# Autodesk Inventor assembly: Shear 1 Assembly
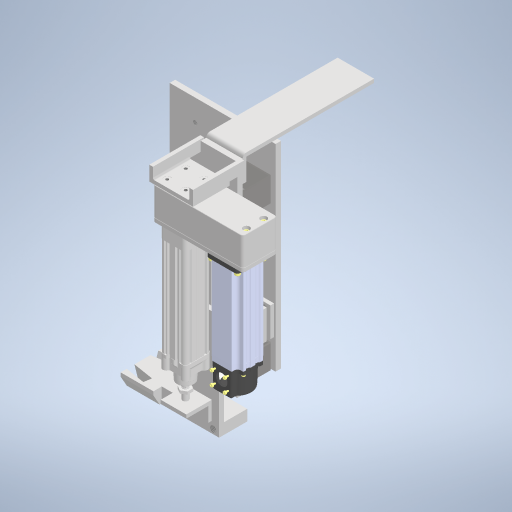
[picture p0: Inventor's stored thumbnail of the model, 512x512]
Saved by Autodesk Inventor 2024.2 (Build 282272000, 272)
## iProperties
Created: 2024-06-10
Part Number: Shear 1 Assembly
Document SubType Name: Assembly
Designer: AC91384
Author: AC91384
## Documents named in this file (12)
- K:\cadlib\1410\43A41410-2557\43A41410-2557.iam
- K:\cadlib\1410\43A41410-2557\Parts\Parts and Drawings\43A41410-2557a.ipt
- K:\cadlib\1410\43A41410-2557\Parts\Parts and Drawings\43A41410-2557B.ipt
- K:\cadlib\1410\43A41410-2557\Parts\Parts and Drawings\43A41410-2557D.ipt
- K:\cadlib\1410\43A41410-2557\Parts\Parts and Drawings\43A41410-2557C.ipt
- K:\cadlib\1410\43A41410-2557\Parts\Parts and Drawings\43A41410-2557Z.iam
- K:\cadlib\1410\43A41410-2557\Parts\Parts and Drawings\43A41410-2557I.ipt
- K:\cadlib\1410\43A41410-2557\Parts\Parts and Drawings\43A41410-2557H.ipt
- K:\cadlib\1410\43A41410-2557\Parts\Parts and Drawings\43A41410-2557F.ipt
- K:\cadlib\1410\43A41410-2557\Parts\Parts and Drawings\43A41410-2557E.ipt
- K:\cadlib\1410\43A41410-2557\Parts\Parts and Drawings\43A41410-2557G.ipt
- K:\cadlib\1410\43A41410-2557\Parts\Parts and Drawings\43A41410-2557J.ipt
## Components (12 placed, 11 different names)
1. 43A41410-2557a:1 — Mate:5, Flush:9, Flush:10, Flush:11, Mate:8, Mate:9, Flush:15, Mate:12, Flush:16, Mate:16, Flush:19, Mate:17, Flush:20
2. 43A41410-2557B:1 — Flush:3, Flush:4, Flush:5, Flush:6, Flush:7, Mate:2, Flush:8, Mate:4, Mate:15
3. 43A41410-2557D:1 — Flush:6, Flush:7, Mate:15
4. 43A41410-2557C:1 — Flush:3, Flush:4, Flush:5
5. 43A41410-2557Z:1 [sub-assembly] — Mate:2, Rotational:1
6. 43A41410-2557I:1 — Flush:8, Mate:4, Mate:5, Flush:9, Flush:10, Mate:11, Mate:14, Flush:18, Flush:21, Flush:22, Flush:23
7. 43A41410-2557H:1 — Flush:14, Mate:9, Flush:15
8. 43A41410-2557H:4 — Flush:11, Mate:8, Flush:14, Flush:23
9. 43A41410-2557F:1 — Mate:11, Rotational:1, Flush:21
10. 43A41410-2557E:1 — Mate:12, Flush:16, Flush:20
11. 43A41410-2557G:1 — Mate:14, Flush:18, Flush:22
12. 43A41410-2557J:1 — Mate:16, Flush:19, Mate:17
## Relationships (30: Flush 18, Mate 11, RevoluteJoint 1)
- Flush:3: 43A41410-2557B:1 ↔ 43A41410-2557C:1
- Flush:4 (19.05 mm): 43A41410-2557B:1 ↔ 43A41410-2557C:1
- Flush:5 (12.7 mm): 43A41410-2557B:1 ↔ 43A41410-2557C:1
- Flush:6: 43A41410-2557B:1 ↔ 43A41410-2557D:1
- Flush:7: 43A41410-2557B:1 ↔ 43A41410-2557D:1
- Mate:2: 43A41410-2557B:1 ↔ 43A41410-2557Z:1
- Flush:8: 43A41410-2557B:1 ↔ 43A41410-2557I:1
- Mate:4 (23.241 mm): 43A41410-2557B:1 ↔ 43A41410-2557I:1
- Mate:5 (50.8 mm): 43A41410-2557a:1 ↔ 43A41410-2557I:1
- Flush:9 (-6.35 mm): 43A41410-2557a:1 ↔ 43A41410-2557I:1
- Flush:10: 43A41410-2557a:1 ↔ 43A41410-2557I:1
- Flush:11 (6.35 mm): 43A41410-2557a:1 ↔ 43A41410-2557H:4
- Mate:8: 43A41410-2557a:1 ↔ 43A41410-2557H:4
- Flush:14: 43A41410-2557H:1 ↔ 43A41410-2557H:4
- Mate:9: 43A41410-2557a:1 ↔ 43A41410-2557H:1
- Flush:15 (50.8 mm): 43A41410-2557a:1 ↔ 43A41410-2557H:1
- Mate:11: 43A41410-2557I:1 ↔ 43A41410-2557F:1
- Rotational:1 [RevoluteJoint]: 43A41410-2557Z:1 ↔ 43A41410-2557F:1
- Mate:12: 43A41410-2557a:1 ↔ 43A41410-2557E:1
- Flush:16 (2.54 mm): 43A41410-2557a:1 ↔ 43A41410-2557E:1
- Mate:14: 43A41410-2557I:1 ↔ 43A41410-2557G:1
- Flush:18 (6.35 mm): 43A41410-2557I:1 ↔ 43A41410-2557G:1
- Mate:15: 43A41410-2557B:1 ↔ 43A41410-2557D:1
- Mate:16: 43A41410-2557a:1 ↔ 43A41410-2557J:1
- Flush:19 (63.5 mm): 43A41410-2557a:1 ↔ 43A41410-2557J:1
- Mate:17 (-57.15 mm): 43A41410-2557a:1 ↔ 43A41410-2557J:1
- Flush:20 (50.8 mm): 43A41410-2557a:1 ↔ 43A41410-2557E:1
- Flush:21 (2.54 mm): 43A41410-2557I:1 ↔ 43A41410-2557F:1
- Flush:22: 43A41410-2557I:1 ↔ 43A41410-2557G:1
- Flush:23 (12.7 mm): 43A41410-2557I:1 ↔ 43A41410-2557H:4
